# Autodesk Inventor assembly: DART Assy
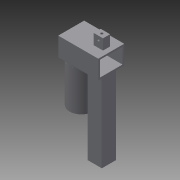
[picture p0: Inventor's stored thumbnail of the model, 180x180]
Saved by Autodesk Inventor 2015 (Build 190159000, 159)
## iProperties
Created: 2015-02-14
Part Number: DART Assy
Document SubType Name: Assembly
Designer: pltwe4
Author: pltwe4
## Documents named in this file (3)
- C:\Users\pltwe4\Documents\recycling-rush\model\DART Assy.iam
- C:\Users\pltwe4\Documents\recycling-rush\model\DART Actuator.ipt
- C:\Users\pltwe4\Documents\recycling-rush\model\CIM motor.ipt
## Components (2 placed, 2 different names)
1. DART Actuator:1 — Mate:2, Mate:3
2. CIM motor:1 — Mate:2, Mate:3
## Relationships (2: Mate 2)
- Mate:2: DART Actuator:1 ↔ CIM motor:1
- Mate:3: DART Actuator:1 ↔ CIM motor:1
